# Autodesk Inventor assembly: Assembly (midterm)
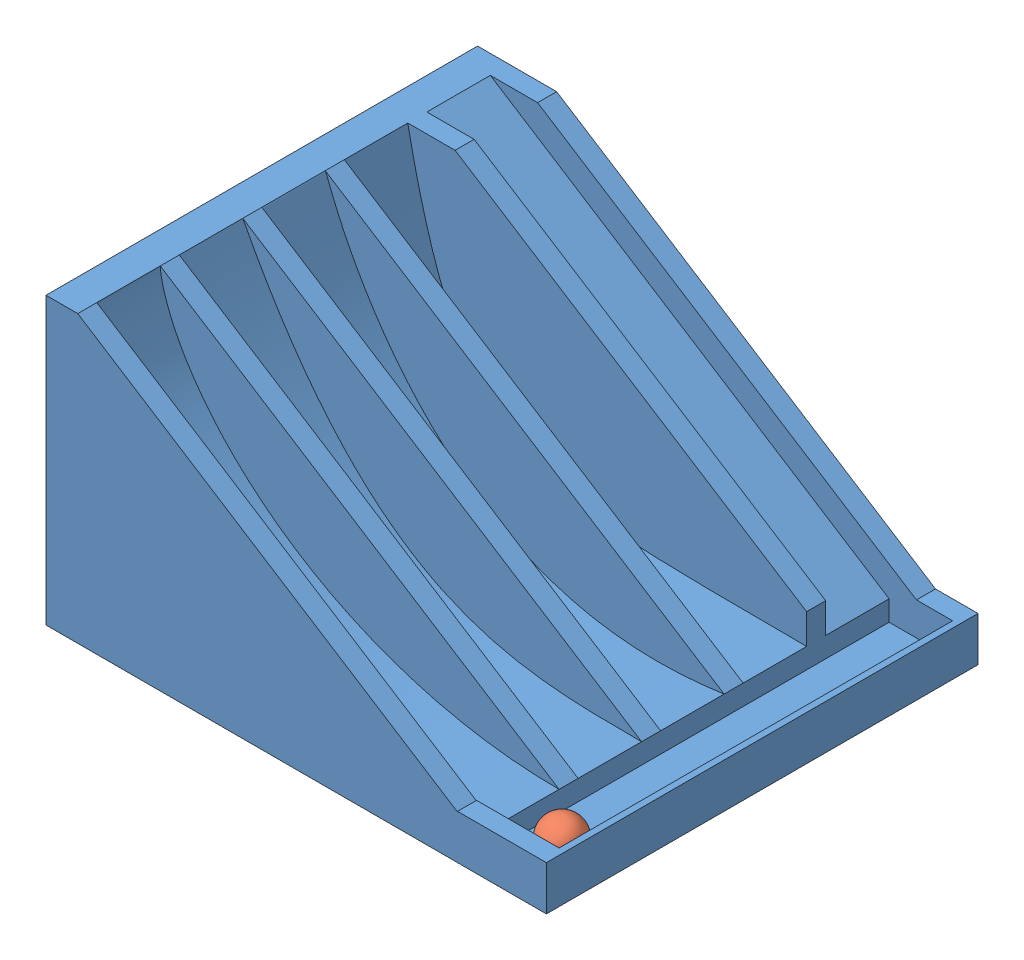
[picture p0: shaded view drawn from the part files that the assembly names]
Saved by Autodesk Inventor 2026.2 (Build 302298010, 298A)
## iProperties
Created: 2026-03-12
Part Number: Assembly (midterm)
Document SubType Name: Assembly
Designer: pjrah
Author: pjrah
## Documents named in this file (9)
- C:\Users\pjrah\Documents\Classes\Spring '26 Classes\PHYS 4003 - Classical Mechanics\Engineering Project\Classical-Mechanics-Project-TU-Sp26\3d_models\Model and Outputs\Assembly (midterm).iam
- C:\Users\pjrah\Documents\Classes\Spring '26 Classes\PHYS 4003 - Classical Mechanics\Engineering Project\Classical-Mechanics-Project-TU-Sp26\3d_models\Model and Outputs\3D Brachistochrone Model (midterm).ipt
- C:\Users\pjrah\Documents\Classes\Spring '26 Classes\PHYS 4003 - Classical Mechanics\Engineering Project\Classical-Mechanics-Project-TU-Sp26\3d_models\Model and Outputs\Glass Marble.ipt
- C:\Users\pjrah\Documents\Classes\Spring '26 Classes\PHYS 4003 - Classical Mechanics\Engineering Project\Classical-Mechanics-Project-TU-Sp26\3d_models\Model and Outputs\Assembly (midterm)\AIP\FEA\fd7kkb6kg.fins
- C:\Users\pjrah\Documents\Classes\Spring '26 Classes\PHYS 4003 - Classical Mechanics\Engineering Project\Classical-Mechanics-Project-TU-Sp26\3d_models\Model and Outputs\Assembly (midterm)\AIP\FEA\fd7kkb6lc.fsat
- C:\Users\pjrah\Documents\Classes\Spring '26 Classes\PHYS 4003 - Classical Mechanics\Engineering Project\Classical-Mechanics-Project-TU-Sp26\3d_models\Model and Outputs\Assembly (midterm)\AIP\FEA\fd7kkb6lc.ftes
- C:\Users\pjrah\Documents\Classes\Spring '26 Classes\PHYS 4003 - Classical Mechanics\Engineering Project\Classical-Mechanics-Project-TU-Sp26\3d_models\Model and Outputs\Assembly (midterm)\AIP\FEA\fd7kkb6lc.fwiz
- C:\Users\pjrah\Documents\Classes\Spring '26 Classes\PHYS 4003 - Classical Mechanics\Engineering Project\Classical-Mechanics-Project-TU-Sp26\3d_models\Model and Outputs\Assembly (midterm)\AIP\FEA\fd7kkb6m8.fmsh
- C:\Users\pjrah\Documents\Classes\Spring '26 Classes\PHYS 4003 - Classical Mechanics\Engineering Project\Classical-Mechanics-Project-TU-Sp26\3d_models\Model and Outputs\Assembly (midterm)\AIP\FEA\fd7kkb6m9.fres
## Components (2 placed, 2 different names)
1. 3D Brachistochrone Model (midterm):1
2. Glass Marble:1
## Named parameters: sa_0 = 25.655
note: some values were not read from the file. Shown as the stored number, unit unknown: "sa_0".
